# Autodesk Inventor assembly: PostLensHolder_B1S_PLS2in
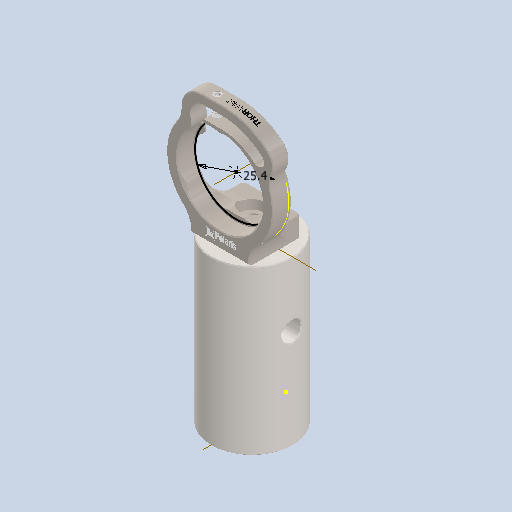
[picture p0: Inventor's stored thumbnail of the model, 512x512]
Saved by Autodesk Inventor 2025.2 (Build 292293000, 293)
## iProperties
Created: 2023-10-19
Part Number: PostLensHolder_B1S_PLS2in
Document SubType Name: Assembly
Designer: S227943
Author: S227943
## Documents named in this file (3)
- C:\Users\monolithic\Documents\GitHub\CAD\Monolith\John\Altair_PowellBaseplate_SPIM_ASLM_CTASLM\Assembly\SubAssemblies\PostLensHolder_B1S_PLS2in.iam
- C:\Users\monolithic\Documents\GitHub\CAD\Monolith\John\Altair_PowellBaseplate_SPIM_ASLM_CTASLM\Assembly\SubAssemblies\POLARIS-B1S-1inOptics.ipt
- C:\Users\monolithic\Documents\GitHub\CAD\Monolith\John\Altair_PowellBaseplate_SPIM_ASLM_CTASLM\Assembly\SubAssemblies\PLS-P2-1inPost2inTall.ipt
## Components (2 placed, 2 different names)
1. POLARIS-B1S-1inOptics:1 — Mate:2, Mate:3
2. PLS-P2-1inPost2inTall:1 — Mate:2, Mate:3
## Relationships (2: Mate 2)
- Mate:2: POLARIS-B1S-1inOptics:1 ↔ PLS-P2-1inPost2inTall:1
- Mate:3: POLARIS-B1S-1inOptics:1 ↔ PLS-P2-1inPost2inTall:1
